# Autodesk Inventor assembly: Assembly
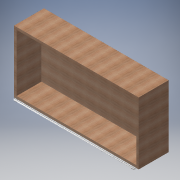
[picture p0: Inventor's stored thumbnail of the model, 180x180]
Saved by Autodesk Inventor 2017 (Build 210142000, 142)
## iProperties
Created: 2016-12-12
Part Number: Assembly
Document SubType Name: Assembly
Designer: umr
Author: umr
## Documents named in this file (9)
- D:\SeniorProject\Models2\Assembly.iam
- D:\SeniorProject\Models2\Base.ipt
- D:\SeniorProject\Models2\BedTrack.ipt
- D:\SeniorProject\Models2\Track Corner Plate.ipt
- D:\SeniorProject\Models2\Wood Screw 99136A600.ipt
- D:\SeniorProject\Models2\M5 Screw with Tee Nut\M5 Screw with Tee Nut.iam
- D:\SeniorProject\Models2\Track Corner Plate_MIR.ipt
- D:\SeniorProject\Models2\Wood Screw 99136A600_MIR.ipt
- D:\SeniorProject\Models2\M5 Screw with Tee Nut\M5 Screw with Tee Nut_MIR.iam
## Components (14 placed, 8 different names)
1. Base:1 — Mate:1, Mate:2, Mate:3, Mate:20, Mate:21, Mate:22
2. BedTrack:1 — Mate:10, Flush:1, Mate:11, Mate:23
3. Track Corner Plate:1 — Mate:1, Mate:2, Mate:3, Cylindrical:1, Cylindrical:2, Mate:4, Mate:5, Mate:6, Mate:7, Mate:8, Mate:9, Flush:1, Mate:11
4. Wood Screw 99136A600:1 — Cylindrical:1
5. Wood Screw 99136A600:2 — Cylindrical:2
6. M5 Screw with Tee Nut:1 [sub-assembly] — Mate:8, Mate:9, Mate:10
7. M5 Screw with Tee Nut:2 [sub-assembly] — Mate:4, Mate:5
8. M5 Screw with Tee Nut:3 [sub-assembly] — Mate:6, Mate:7
9. Track Corner Plate_MIR:1 — Mate:14, Mate:15, Mate:16, Mate:17, Mate:18, Mate:19, Cylindrical:3, Cylindrical:4, Mate:20
10. Wood Screw 99136A600_MIR:1 — Cylindrical:3, Mate:21
11. Wood Screw 99136A600_MIR:2 — Cylindrical:4, Mate:22
12. M5 Screw with Tee Nut_MIR:1 [sub-assembly] — Mate:14, Mate:15, Mate:23
13. M5 Screw with Tee Nut_MIR:2 [sub-assembly] — Mate:16, Mate:17
14. M5 Screw with Tee Nut_MIR:3 [sub-assembly] — Mate:18, Mate:19
## Relationships (26: Mate 21, CylindricalJoint 4, Flush 1)
- Mate:1: Base:1 ↔ Track Corner Plate:1
- Mate:2: Base:1 ↔ Track Corner Plate:1
- Mate:3: Base:1 ↔ Track Corner Plate:1
- Cylindrical:1: Track Corner Plate:1 ↔ Wood Screw 99136A600:1
- Cylindrical:2: Track Corner Plate:1 ↔ Wood Screw 99136A600:2
- Mate:4: Track Corner Plate:1 ↔ M5 Screw with Tee Nut:2
- Mate:5: Track Corner Plate:1 ↔ M5 Screw with Tee Nut:2
- Mate:6: Track Corner Plate:1 ↔ M5 Screw with Tee Nut:3
- Mate:7: Track Corner Plate:1 ↔ M5 Screw with Tee Nut:3
- Mate:8: Track Corner Plate:1 ↔ M5 Screw with Tee Nut:1
- Mate:9: Track Corner Plate:1 ↔ M5 Screw with Tee Nut:1
- Mate:10: BedTrack:1 ↔ M5 Screw with Tee Nut:1
- Flush:1 (-8 mm): BedTrack:1 ↔ Track Corner Plate:1
- Mate:11: BedTrack:1 ↔ Track Corner Plate:1
- Mate:14: Track Corner Plate_MIR:1 ↔ M5 Screw with Tee Nut_MIR:1
- Mate:15: Track Corner Plate_MIR:1 ↔ M5 Screw with Tee Nut_MIR:1
- Mate:16: Track Corner Plate_MIR:1 ↔ M5 Screw with Tee Nut_MIR:2
- Mate:17: Track Corner Plate_MIR:1 ↔ M5 Screw with Tee Nut_MIR:2
- Mate:18: Track Corner Plate_MIR:1 ↔ M5 Screw with Tee Nut_MIR:3
- Mate:19: Track Corner Plate_MIR:1 ↔ M5 Screw with Tee Nut_MIR:3
- Cylindrical:3: Track Corner Plate_MIR:1 ↔ Wood Screw 99136A600_MIR:1
- Cylindrical:4: Track Corner Plate_MIR:1 ↔ Wood Screw 99136A600_MIR:2
- Mate:20: Base:1 ↔ Track Corner Plate_MIR:1
- Mate:21: Base:1 ↔ Wood Screw 99136A600_MIR:1
- Mate:22: Base:1 ↔ Wood Screw 99136A600_MIR:2
- Mate:23: BedTrack:1 ↔ M5 Screw with Tee Nut_MIR:1
